# Autodesk Inventor assembly: smallest robot manuplator
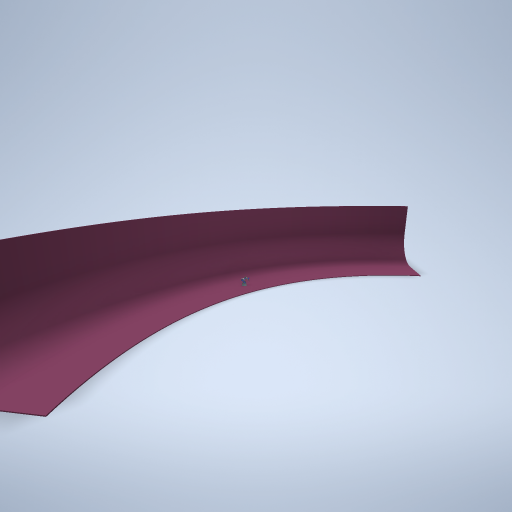
[picture p0: Inventor's stored thumbnail of the model, 512x512]
Saved by Autodesk Inventor 2023.2 (Build 272271000, 271)
## iProperties
Created: 2022-12-18
Part Number: smallest robot manuplator
Document SubType Name: Assembly
Designer: omrfrkmll
Author: omrfrkmll
## Documents named in this file (12)
- C:\Users\omr_f\Desktop\smallest robot manuplator\smallest robot manuplator.iam
- C:\Users\omr_f\Desktop\smallest robot manuplator\A.ipt
- C:\Users\omr_f\Desktop\smallest robot manuplator\B ufak servo.ipt
- C:\Users\omr_f\Desktop\smallest robot manuplator\SG90_Model_A.ipt
- C:\Users\omr_f\Desktop\smallest robot manuplator\firsarm.ipt
- C:\Users\omr_f\Desktop\smallest robot manuplator\secondlink.ipt
- C:\Users\omr_f\Desktop\smallest robot manuplator\sg90-servomotor-1.snapshot.32\SG90_Arm_04_Custom\SG90_Arm_04_Custom\SG90_Arm_04_Custom.ipt
- C:\Users\omr_f\Desktop\smallest robot manuplator\endeffectortutucu.ipt
- C:\Users\omr_f\Desktop\smallest robot manuplator\endeffector.ipt
- C:\Users\omr_f\Desktop\smallest robot manuplator\gripper.ipt
- C:\Users\omr_f\Desktop\smallest robot manuplator\gripper_MIR.ipt
- C:\Users\omr_f\Desktop\smallest robot manuplator\baase.ipt
## Components (21 placed, 11 different names)
1. A:1 — Mate:7, Mate:8, Mate:24, Mate:33, Mate:34, Mate:79
2. B ufak servo:1 — Mate:7, Mate:8, Mate:9, Mate:10, Mate:11, Mate:28
3. SG90_Model_A:1 — Mate:9, Mate:10, Mate:11, Mate:12, Mate:31, Mate:32
4. firsarm:1 — Mate:12, Mate:14, Mate:36, Mate:37, Mate:39, Mate:40, Mate:56
5. SG90_Model_A:2 — Mate:14, Mate:29, Mate:36, Mate:37, Mate:38, Mate:40
6. secondlink:1 — Mate:21, Mate:41, Mate:42, Mate:43, Mate:44, Mate:55
7. SG90_Model_A:3 — Mate:21, Mate:43, Mate:44, Mate:45, Mate:46, Mate:48
8. SG90_Model_A:4 — Mate:24, Mate:26, Mate:27, Mate:33, Mate:34
9. SG90_Arm_04_Custom:1 — Mate:26, Mate:27, Mate:28
10. SG90_Arm_04_Custom:2 — Mate:29, Mate:38, Mate:41, Mate:42, Mate:55
11. SG90_Arm_04_Custom:3 — Mate:31, Mate:32, Mate:39, Mate:56
12. SG90_Arm_04_Custom:4 — Mate:45, Mate:46, Mate:47, Mate:50
13. endeffectortutucu:1 — Mate:47, Mate:48, Mate:49, Flush:1, Mate:50, Mate:51, Mate:52
14. SG90_Model_A:5 — Mate:49, Flush:1, Mate:51, Mate:52, Mate:53, Mate:54, Mate:57
15. SG90_Arm_04_Custom:5 — Mate:53, Mate:54, Mate:58, Flush:2
16. endeffector:1 — Mate:57, Mate:58, Flush:2, Mate:60, Mate:61, Flush:3, Mate:72, Mate:74, Mate:78
17. SG90_Model_A:6 — Mate:60, Mate:61, Flush:3, Mate:63, Mate:64
18. SG90_Arm_04_Custom:6 — Mate:63, Mate:64, Mate:71, Mate:73
19. gripper:1 — Mate:71, Mate:73
20. gripper_MIR:1 — Mate:72, Mate:74, Mate:78
21. baase:1 — Mate:79, Mate:80
## Relationships (54: Mate 51, Flush 3)
- Mate:7: A:1 ↔ B ufak servo:1
- Mate:8: A:1 ↔ B ufak servo:1
- Mate:9: B ufak servo:1 ↔ SG90_Model_A:1
- Mate:10: B ufak servo:1 ↔ SG90_Model_A:1
- Mate:11: B ufak servo:1 ↔ SG90_Model_A:1
- Mate:12: SG90_Model_A:1 ↔ firsarm:1
- Mate:14: firsarm:1 ↔ SG90_Model_A:2
- Mate:21: secondlink:1 ↔ SG90_Model_A:3
- Mate:24: A:1 ↔ SG90_Model_A:4
- Mate:26: SG90_Model_A:4 ↔ SG90_Arm_04_Custom:1
- Mate:27: SG90_Model_A:4 ↔ SG90_Arm_04_Custom:1
- Mate:28: B ufak servo:1 ↔ SG90_Arm_04_Custom:1
- Mate:29: SG90_Model_A:2 ↔ SG90_Arm_04_Custom:2
- Mate:31: SG90_Model_A:1 ↔ SG90_Arm_04_Custom:3
- Mate:32: SG90_Model_A:1 ↔ SG90_Arm_04_Custom:3
- Mate:33: A:1 ↔ SG90_Model_A:4
- Mate:34: A:1 ↔ SG90_Model_A:4
- Mate:36: firsarm:1 ↔ SG90_Model_A:2
- Mate:37: firsarm:1 ↔ SG90_Model_A:2
- Mate:38: SG90_Model_A:2 ↔ SG90_Arm_04_Custom:2
- Mate:39: firsarm:1 ↔ SG90_Arm_04_Custom:3
- Mate:40: firsarm:1 ↔ SG90_Model_A:2
- Mate:41: secondlink:1 ↔ SG90_Arm_04_Custom:2
- Mate:42: secondlink:1 ↔ SG90_Arm_04_Custom:2
- Mate:43: secondlink:1 ↔ SG90_Model_A:3
- Mate:44: secondlink:1 ↔ SG90_Model_A:3
- Mate:45: SG90_Model_A:3 ↔ SG90_Arm_04_Custom:4
- Mate:46: SG90_Model_A:3 ↔ SG90_Arm_04_Custom:4
- Mate:47: SG90_Arm_04_Custom:4 ↔ endeffectortutucu:1
- Mate:48: SG90_Model_A:3 ↔ endeffectortutucu:1
- Mate:49: endeffectortutucu:1 ↔ SG90_Model_A:5
- Flush:1: endeffectortutucu:1 ↔ SG90_Model_A:5
- Mate:50: SG90_Arm_04_Custom:4 ↔ endeffectortutucu:1
- Mate:51: endeffectortutucu:1 ↔ SG90_Model_A:5
- Mate:52: endeffectortutucu:1 ↔ SG90_Model_A:5
- Mate:53: SG90_Model_A:5 ↔ SG90_Arm_04_Custom:5
- Mate:54: SG90_Model_A:5 ↔ SG90_Arm_04_Custom:5
- Mate:55: secondlink:1 ↔ SG90_Arm_04_Custom:2
- Mate:56: firsarm:1 ↔ SG90_Arm_04_Custom:3
- Mate:57: SG90_Model_A:5 ↔ endeffector:1
- Mate:58: SG90_Arm_04_Custom:5 ↔ endeffector:1
- Flush:2: SG90_Arm_04_Custom:5 ↔ endeffector:1
- Mate:60: endeffector:1 ↔ SG90_Model_A:6
- Mate:61: endeffector:1 ↔ SG90_Model_A:6
- Flush:3: endeffector:1 ↔ SG90_Model_A:6
- Mate:63: SG90_Model_A:6 ↔ SG90_Arm_04_Custom:6
- Mate:64: SG90_Model_A:6 ↔ SG90_Arm_04_Custom:6
- Mate:71: SG90_Arm_04_Custom:6 ↔ gripper:1
- Mate:72: endeffector:1 ↔ gripper_MIR:1
- Mate:73: SG90_Arm_04_Custom:6 ↔ gripper:1
- Mate:74: endeffector:1 ↔ gripper_MIR:1
- Mate:78: endeffector:1 ↔ gripper_MIR:1
- Mate:79: A:1 ↔ baase:1
- Mate:80: baase:1
